# Autodesk Inventor assembly: pcb_assembled_2
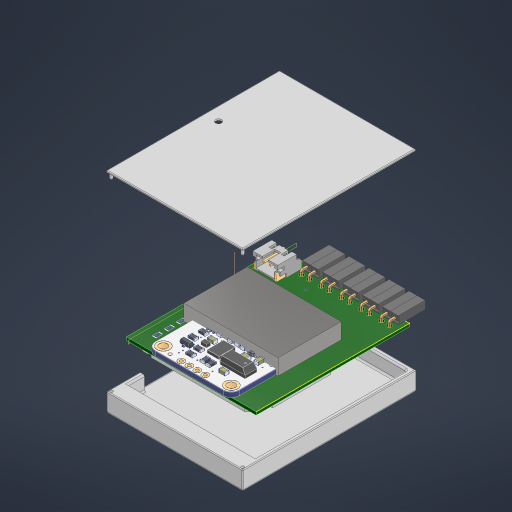
[picture p0: Inventor's stored thumbnail of the model, 512x512]
Saved by Autodesk Inventor 2023 (Build 270158000, 158)
## iProperties
Created: 2022-04-29
Part Number: pcb_assembled_2
Document SubType Name: Assembly
Designer: Haroon Nawaz
Author: Haroon Nawaz
## Documents named in this file (5)
- C:\Users\Haroon Nawaz\Documents\1_Haroon\CE347\git\CE347_Gest\hardware\3D_CAD\pcb_assembled_2.iam
- C:\Users\Haroon Nawaz\Documents\1_Haroon\CE347\git\CE347_Gest\hardware\3D_CAD\pcb_assembled.iam
- C:\Users\Haroon Nawaz\Documents\1_Haroon\CE347\git\CE347_Gest\hardware\3D_CAD\enclosure2.ipt
- C:\Users\Haroon Nawaz\Documents\1_Haroon\CE347\git\CE347_Gest\hardware\3D_CAD\battery.ipt
- C:\Users\Haroon Nawaz\Documents\1_Haroon\CE347\git\CE347_Gest\hardware\3D_CAD\enclosure_lid.ipt
## Components (4 placed, 4 different names)
1. pcb_assembled:1 [sub-assembly] — Mate:1, Mate:2, Mate:3
2. enclosure2:1 — Mate:1, Mate:2, Mate:4
3. battery:1 — Mate:3
4. enclosure_lid:1 — Mate:4
## Relationships (4: Mate 4)
- Mate:1 (1.27 mm): pcb_assembled:1 ↔ enclosure2:1
- Mate:2: pcb_assembled:1 ↔ enclosure2:1
- Mate:3: pcb_assembled:1 ↔ battery:1
- Mate:4: enclosure2:1 ↔ enclosure_lid:1
